# Autodesk Inventor assembly: 1 Presentation Assembly
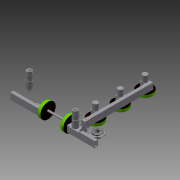
[picture p0: Inventor's stored thumbnail of the model, 180x180]
Saved by Autodesk Inventor 2015 (Build 190159000, 159)
## iProperties
Created: 2015-01-27
Part Number: 1 Presentation Assembly
Document SubType Name: Assembly
Designer: chapale16
Author: chapale16
## Documents named in this file (9)
- \\lhssvr02\Homedirs\Robotics Club\CAD Model 2015\CDR prep\Tote Collector Arms\1 Presentation Assembly.iam
- \\lhssvr02\Homedirs\Robotics Club\CAD Model 2015\CDR prep\Tote Collector Arms\Frame.ipt
- \\lhssvr02\Homedirs\Robotics Club\CAD Model 2015\CDR prep\Tote Collector Arms\Right side collector assembly_MIR1.iam
- \\lhssvr02\Homedirs\Robotics Club\CAD Model 2015\Front bar with Motors.iam
- \\lhssvr02\Homedirs\Robotics Club\CAD Model 2015\CDR prep\Tote Collector Arms\collector arm wheel.ipt
- \\lhssvr02\Homedirs\Robotics Club\CAD Model 2015\CDR prep\Tote Collector Arms\collector Axle.ipt
- \\lhssvr02\Homedirs\Robotics Club\CAD Model 2015\Modified Front Frame 27 in.ipt
- \\lhssvr02\Homedirs\Robotics Club\CAD Model 2015\1.5 in bearing block.ipt
- \\lhssvr02\Homedirs\Robotics Club\CAD Model 2015\CDR prep\Tote Collector Arms\PG-71-am-0914.ipt
## Components (8 placed, 8 different names)
1. Frame:1 — Mate:3, Angle:1, Mate:5, Flush:1
2. Right side collector assembly_MIR1:1 [sub-assembly] — Mate:3
3. Front bar with Motors:1 [sub-assembly] — Angle:1, Mate:5, Flush:1, Mate:6, Mate:7, Mate:8, Mate:9, Flush:2, Flush:3, Mate:12
4. collector arm wheel:1 — Mate:6, Mate:7, Mate:10
5. collector Axle:1 — Mate:8, Mate:9, Mate:11, Mate:12
6. Modified Front Frame 27 in:1 — Mate:10, Flush:2, Flush:3, Angle:2
7. 1.5 in bearing block:1 — Mate:11, Angle:2
8. PG-71-am-0914:1
## Relationships (14: Mate 9, Flush 3, Angle 2)
- Mate:3: Frame:1 ↔ Right side collector assembly_MIR1:1
- Angle:1 (180 deg): Frame:1 ↔ Front bar with Motors:1
- Mate:5: Frame:1 ↔ Front bar with Motors:1
- Flush:1: Frame:1 ↔ Front bar with Motors:1
- Mate:6 (165.1 mm): Front bar with Motors:1 ↔ collector arm wheel:1
- Mate:7: Front bar with Motors:1 ↔ collector arm wheel:1
- Mate:8: Front bar with Motors:1 ↔ collector Axle:1
- Mate:9: Front bar with Motors:1 ↔ collector Axle:1
- Mate:10 (12.7 mm): collector arm wheel:1 ↔ Modified Front Frame 27 in:1
- Flush:2: Front bar with Motors:1 ↔ Modified Front Frame 27 in:1
- Flush:3: Front bar with Motors:1 ↔ Modified Front Frame 27 in:1
- Mate:11: collector Axle:1 ↔ 1.5 in bearing block:1
- Angle:2 (0 deg): Modified Front Frame 27 in:1 ↔ 1.5 in bearing block:1
- Mate:12: Front bar with Motors:1 ↔ collector Axle:1
